# Autodesk Inventor assembly: BatteryPack
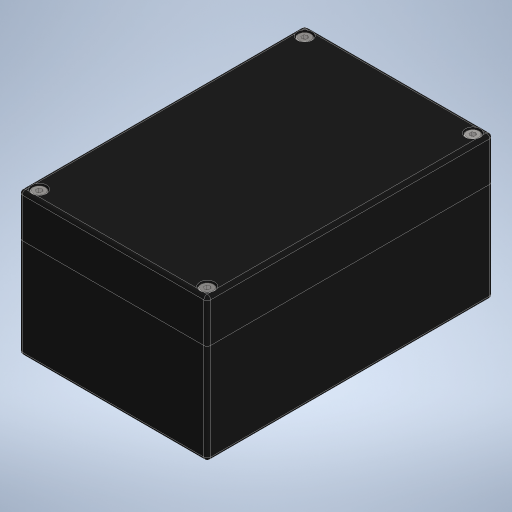
[picture p0: Inventor's stored thumbnail of the model, 512x512]
Saved by Autodesk Inventor 2024 (Build 280153000, 153)
## iProperties
Created: 2023-12-27
Part Number: BatteryPack
Document SubType Name: Assembly
Designer: denni
Author: denni
## Documents named in this file (7)
- D:\GIT\ThreadedInsertPress\Parts\BatteryPack.iam
- D:\GIT\ThreadedInsertPress\Parts\3D printed\BatterieClamp.ipt
- D:\GIT\ThreadedInsertPress\Parts\Others\AA Battery\AA Battery.ipt
- D:\GIT\ThreadedInsertPress\Parts\3D printed\BatteryCase_Botton.ipt
- D:\GIT\ThreadedInsertPress\Parts\3D printed\BatteryCase_Top.ipt
- D:\Inventor\Content Center Files\R2024\de-DE\ISO 10642(2)\ISO 10642  - M3  x  10.ipt
- D:\Inventor\Content Center Files\R2024\de-DE\ISO 4762(1)\DIN EN ISO 4762 - M2 x 20.ipt
## Components (17 placed, 6 different names)
1. BatterieClamp:1 — Passend:1, Passend:2, Passend:3, Passend:4, Passend:5, Passend:6, Passend:7, Passend:8
2. AA Battery:1 — Passend:2, Fluchtend:1, Fluchtend:2
3. AA Battery:2 — Passend:4, Fluchtend:3, Fluchtend:4, Passend:11
4. AA Battery:3 — Passend:3, Fluchtend:2, Fluchtend:3
5. AA Battery:4 — Passend:1, Fluchtend:1, Passend:12
6. AA Battery:5 — Passend:5, Fluchtend:7, Passend:10
7. AA Battery:6 — Passend:6, Fluchtend:6, Fluchtend:7
8. AA Battery:7 — Passend:7, Fluchtend:5, Fluchtend:6
9. AA Battery:8 — Passend:8, Fluchtend:4, Fluchtend:5, Passend:9
10. BatteryCase_Botton:1 — Passend:9, Passend:10, Passend:13, Passend:14, Passend:15
11. BatteryCase_Top:1 — Passend:11, Passend:12, Passend:13, Einfügen:1, Einfügen:2, Einfügen:3, Einfügen:4
12. DIN EN ISO 10642 M3  x  10:1 — Passend:14
13. DIN EN ISO 10642 M3  x  10:2 — Passend:15
14. DIN EN ISO 4762 M2 x 20:1 — Einfügen:1
15. DIN EN ISO 4762 M2 x 20:2 — Einfügen:2
16. DIN EN ISO 4762 M2 x 20:3 — Einfügen:3
17. DIN EN ISO 4762 M2 x 20:4 — Einfügen:4
## Relationships (26: Mate 15, Flush 7, Insert 4)
- Passend:1 [Mate]: BatterieClamp:1 ↔ AA Battery:4
- Passend:2 [Mate]: BatterieClamp:1 ↔ AA Battery:1
- Passend:3 [Mate]: BatterieClamp:1 ↔ AA Battery:3
- Passend:4 [Mate]: BatterieClamp:1 ↔ AA Battery:2
- Passend:5 [Mate]: BatterieClamp:1 ↔ AA Battery:5
- Passend:6 [Mate]: BatterieClamp:1 ↔ AA Battery:6
- Passend:7 [Mate]: BatterieClamp:1 ↔ AA Battery:7
- Passend:8 [Mate]: BatterieClamp:1 ↔ AA Battery:8
- Fluchtend:1 [Flush]: AA Battery:1 ↔ AA Battery:4
- Fluchtend:2 [Flush]: AA Battery:1 ↔ AA Battery:3
- Fluchtend:3 [Flush]: AA Battery:2 ↔ AA Battery:3
- Fluchtend:4 [Flush]: AA Battery:2 ↔ AA Battery:8
- Fluchtend:5 [Flush]: AA Battery:7 ↔ AA Battery:8
- Fluchtend:6 [Flush]: AA Battery:6 ↔ AA Battery:7
- Fluchtend:7 [Flush]: AA Battery:5 ↔ AA Battery:6
- Passend:9 [Mate]: AA Battery:8 ↔ BatteryCase_Botton:1
- Passend:10 [Mate]: AA Battery:5 ↔ BatteryCase_Botton:1
- Passend:11 [Mate]: AA Battery:2 ↔ BatteryCase_Top:1
- Passend:12 [Mate]: AA Battery:4 ↔ BatteryCase_Top:1
- Passend:13 [Mate]: BatteryCase_Botton:1 ↔ BatteryCase_Top:1
- Passend:14 [Mate]: BatteryCase_Botton:1 ↔ DIN EN ISO 10642 M3  x  10:1
- Passend:15 [Mate]: BatteryCase_Botton:1 ↔ DIN EN ISO 10642 M3  x  10:2
- Einfügen:1 [Insert]: BatteryCase_Top:1 ↔ DIN EN ISO 4762 M2 x 20:1
- Einfügen:2 [Insert]: BatteryCase_Top:1 ↔ DIN EN ISO 4762 M2 x 20:2
- Einfügen:3 [Insert]: BatteryCase_Top:1 ↔ DIN EN ISO 4762 M2 x 20:3
- Einfügen:4 [Insert]: BatteryCase_Top:1 ↔ DIN EN ISO 4762 M2 x 20:4
